# Autodesk Inventor assembly: 3inch OmniWheel
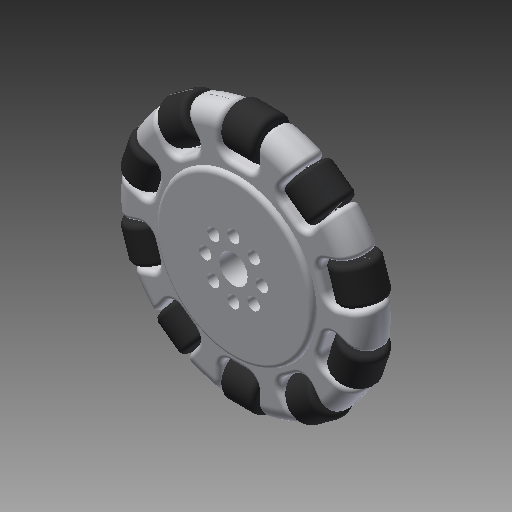
[picture p0: Inventor's stored thumbnail of the model, 512x512]
Saved by Autodesk Inventor 2019 (Build 230136000, 136)
## iProperties
Created: 2012-11-03
Part Number: 3inch OmniWheel
Document SubType Name: Assembly
Designer: Rob
Mass: 39.568 g
Surface Area: 227.376 cm^2
Volume: 39.568 cm^3
Density: 1 g/cm^3
Author: Rob
## Documents named in this file (2)
- C:\Users\Admin\Documents\Inventor\Doan\3inch OmniWheel.iam
- C:\Users\Admin\Documents\Inventor\Doan\3inch OmniWheel.ipt
## Components (2 placed, 1 different names)
1. 3inch OmniWheel:1 — Insert:1
2. 3inch OmniWheel:2 — Insert:1
## Relationships (1: Insert 1)
- Insert:1: 3inch OmniWheel:1 ↔ 3inch OmniWheel:2
